# Autodesk Inventor assembly: Test Section Assembly
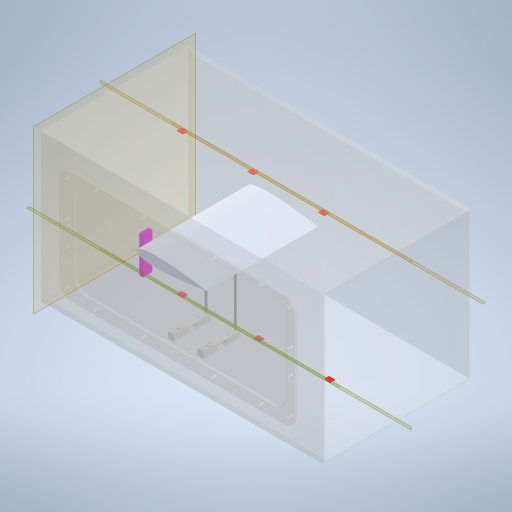
[picture p0: Inventor's stored thumbnail of the model, 512x512]
Saved by Autodesk Inventor 2023 (Build 270158000, 158)
## iProperties
Created: 2022-03-05
Part Number: Test Section Assembly
Document SubType Name: Assembly
Designer: kamer
Author: kamer
## iProperties of the stored document MemberDocs/xAaaaqqaaAaaaaaaaAaaaqncaKc
Created: 2022-03-05
Part Number: Test Section Assembly
Document SubType Name: Assembly
Designer: kamer
Author: kamer
## Documents named in this file (13)
- X:\Storage\Documents\ME 306 Heat Transfer Project Files\CAD\Test Section Assembly.iam
- X:\Storage\Documents\ME 306 Heat Transfer Project Files\CAD\Wind Tunnel Test Section Back.ipt
- X:\Storage\Documents\ME 306 Heat Transfer Project Files\CAD\Wind Tunnel Test Section Bottom.ipt
- X:\Storage\Documents\ME 306 Heat Transfer Project Files\CAD\Wind Tunnel Test Section Front.ipt
- X:\Storage\Documents\ME 306 Heat Transfer Project Files\CAD\Wind Tunnel Test Section Top.ipt
- X:\Storage\Documents\ME 306 Heat Transfer Project Files\CAD\Wind Tunnel Test Section Door Inner.ipt
- X:\Storage\Documents\ME 306 Heat Transfer Project Files\CAD\Wind Tunnel Test Section Door Outer.ipt
- X:\Storage\Documents\ME 306 Heat Transfer Project Files\CAD\Load Cell Spacer.ipt
- X:\Storage\Documents\ME 306 Heat Transfer Project Files\CAD\Mockup Load Cell (based on 1kg Adafruit).ipt
- X:\Storage\Documents\ME 306 Heat Transfer Project Files\CAD\naca0015_airfoil_heatstakes.ipt
- X:\Storage\Documents\ME 306 Heat Transfer Project Files\CAD\4mm threadstock 7in length.ipt
- X:\Storage\Documents\ME 306 Heat Transfer Project Files\CAD\Mockup Barometer.ipt
- X:\Storage\Documents\ME 306 Heat Transfer Project Files\CAD\Mockup Anemometer.ipt
## Components (22 placed, 12 different names)
1. Wind Tunnel Test Section Back:1 — Mate:1, Flush:1, Mate:4, Mate:5, Mate:42
2. Wind Tunnel Test Section Bottom:1 — Mate:1, Flush:1, Mate:2, Flush:2, Mate:10, Mate:15, Mate:16, Mate:21, Mate:22, Mate:23, Mate:35, Mate:36, Mate:37, Mate:38, Mate:39, Mate:40, Mate:41, Flush:14
3. Wind Tunnel Test Section Front:1 — Mate:2, Flush:2, Mate:3, Flush:3, Mate:5, Mate:6, Flush:4, Mate:7, Mate:8, Angle:1, Mate:24, Angle:3, Mate:43
4. Wind Tunnel Test Section Top:1 — Mate:3, Flush:3, Mate:4, Mate:6, Mate:28, Mate:29, Mate:30, Mate:31, Mate:32, Mate:33, Mate:34
5. Wind Tunnel Test Section Door Inner:1 — Flush:4, Mate:7, Mate:8, Mate:9, Flush:5, Flush:6
6. Wind Tunnel Test Section Door Outer:1 — Mate:9, Flush:5, Flush:6
7. Load Cell Spacer:1 — Mate:11, Mate:12, Mate:15
8. Mockup Load Cell (based on 1kg Adafruit):1 — Mate:10, Mate:11, Mate:12, Mate:13, Mate:14, Angle:1, Mate:26, Angle:2
9. Load Cell Spacer:2 — Mate:13, Mate:14
10. Mockup Load Cell (based on 1kg Adafruit):2 — Mate:16, Mate:17, Mate:18, Mate:19, Mate:20, Mate:25, Angle:2
11. Load Cell Spacer:3 — Mate:18, Mate:20, Mate:21
12. Load Cell Spacer:4 — Mate:17, Mate:19
13. naca0015_airfoil_heatstakes:1 — Mate:22, Mate:23, Mate:24, Mate:27
14. 4mm threadstock 7in length:1 — Mate:26, Mate:27, Flush:8
15. 4mm threadstock 7in length:2 — Mate:25, Flush:8
16. Mockup Barometer:1 — Mate:33, Mate:34, Flush:10, Flush:11
17. Mockup Barometer:2 — Mate:36, Mate:37, Flush:12
18. Mockup Barometer:3 — Mate:31, Mate:32, Flush:9, Flush:10, Flush:12
19. Mockup Barometer:4 — Mate:38, Mate:39, Flush:13
20. Mockup Barometer:5 — Mate:28, Mate:29, Mate:30, Flush:9, Flush:13
21. Mockup Barometer:6 — Mate:35, Flush:11, Mate:40
22. Mockup Anemometer:1 — Mate:41, Angle:3, Flush:14, Mate:44
## Relationships (60: Mate 44, Flush 13, Angle 3)
- Mate:1: Wind Tunnel Test Section Back:1 ↔ Wind Tunnel Test Section Bottom:1
- Flush:1: Wind Tunnel Test Section Back:1 ↔ Wind Tunnel Test Section Bottom:1
- Mate:2: Wind Tunnel Test Section Bottom:1 ↔ Wind Tunnel Test Section Front:1
- Flush:2: Wind Tunnel Test Section Bottom:1 ↔ Wind Tunnel Test Section Front:1
- Mate:3: Wind Tunnel Test Section Front:1 ↔ Wind Tunnel Test Section Top:1
- Flush:3: Wind Tunnel Test Section Front:1 ↔ Wind Tunnel Test Section Top:1
- Mate:4: Wind Tunnel Test Section Back:1 ↔ Wind Tunnel Test Section Top:1
- Mate:5 (306.3494 mm): Wind Tunnel Test Section Back:1 ↔ Wind Tunnel Test Section Front:1
- Mate:6: Wind Tunnel Test Section Front:1 ↔ Wind Tunnel Test Section Top:1
- Flush:4: Wind Tunnel Test Section Front:1 ↔ Wind Tunnel Test Section Door Inner:1
- Mate:7: Wind Tunnel Test Section Front:1 ↔ Wind Tunnel Test Section Door Inner:1
- Mate:8: Wind Tunnel Test Section Front:1 ↔ Wind Tunnel Test Section Door Inner:1
- Mate:9: Wind Tunnel Test Section Door Inner:1 ↔ Wind Tunnel Test Section Door Outer:1
- Flush:5 (-26.2763 mm): Wind Tunnel Test Section Door Inner:1 ↔ Wind Tunnel Test Section Door Outer:1
- Flush:6 (-18.2753 mm): Wind Tunnel Test Section Door Inner:1 ↔ Wind Tunnel Test Section Door Outer:1
- Mate:10: Wind Tunnel Test Section Bottom:1 ↔ Mockup Load Cell (based on 1kg Adafruit):1
- Mate:11: Load Cell Spacer:1 ↔ Mockup Load Cell (based on 1kg Adafruit):1
- Mate:12: Load Cell Spacer:1 ↔ Mockup Load Cell (based on 1kg Adafruit):1
- Mate:13: Mockup Load Cell (based on 1kg Adafruit):1 ↔ Load Cell Spacer:2
- Mate:14: Mockup Load Cell (based on 1kg Adafruit):1 ↔ Load Cell Spacer:2
- Mate:15: Wind Tunnel Test Section Bottom:1 ↔ Load Cell Spacer:1
- Angle:1 (270 deg): Wind Tunnel Test Section Front:1 ↔ Mockup Load Cell (based on 1kg Adafruit):1
- Mate:16: Wind Tunnel Test Section Bottom:1 ↔ Mockup Load Cell (based on 1kg Adafruit):2
- Mate:17: Mockup Load Cell (based on 1kg Adafruit):2 ↔ Load Cell Spacer:4
- Mate:18: Mockup Load Cell (based on 1kg Adafruit):2 ↔ Load Cell Spacer:3
- Mate:19: Mockup Load Cell (based on 1kg Adafruit):2 ↔ Load Cell Spacer:4
- Mate:20: Mockup Load Cell (based on 1kg Adafruit):2 ↔ Load Cell Spacer:3
- Mate:21: Wind Tunnel Test Section Bottom:1 ↔ Load Cell Spacer:3
- Mate:22: Wind Tunnel Test Section Bottom:1 ↔ naca0015_airfoil_heatstakes:1
- Mate:23: Wind Tunnel Test Section Bottom:1 ↔ naca0015_airfoil_heatstakes:1
- Mate:24: Wind Tunnel Test Section Front:1 ↔ naca0015_airfoil_heatstakes:1
- Mate:25: Mockup Load Cell (based on 1kg Adafruit):2 ↔ 4mm threadstock 7in length:2
- Mate:26: Mockup Load Cell (based on 1kg Adafruit):1 ↔ 4mm threadstock 7in length:1
- Mate:27: naca0015_airfoil_heatstakes:1 ↔ 4mm threadstock 7in length:1
- Flush:8: 4mm threadstock 7in length:1 ↔ 4mm threadstock 7in length:2
- Mate:28: Wind Tunnel Test Section Top:1 ↔ Mockup Barometer:5
- Mate:29: Wind Tunnel Test Section Top:1 ↔ Mockup Barometer:5
- Mate:30 (-5 mm): Wind Tunnel Test Section Top:1 ↔ Mockup Barometer:5
- Mate:31: Wind Tunnel Test Section Top:1 ↔ Mockup Barometer:3
- Mate:32: Wind Tunnel Test Section Top:1 ↔ Mockup Barometer:3
- Flush:9: Mockup Barometer:3 ↔ Mockup Barometer:5
- Mate:33: Wind Tunnel Test Section Top:1 ↔ Mockup Barometer:1
- Mate:34: Wind Tunnel Test Section Top:1 ↔ Mockup Barometer:1
- Flush:10: Mockup Barometer:1 ↔ Mockup Barometer:3
- Angle:2 (180 deg): Mockup Load Cell (based on 1kg Adafruit):1 ↔ Mockup Load Cell (based on 1kg Adafruit):2
- Mate:35: Wind Tunnel Test Section Bottom:1 ↔ Mockup Barometer:6
- Flush:11: Mockup Barometer:1 ↔ Mockup Barometer:6
- Mate:36: Wind Tunnel Test Section Bottom:1 ↔ Mockup Barometer:2
- Mate:37: Wind Tunnel Test Section Bottom:1 ↔ Mockup Barometer:2
- Flush:12: Mockup Barometer:2 ↔ Mockup Barometer:3
- Mate:38: Wind Tunnel Test Section Bottom:1 ↔ Mockup Barometer:4
- Mate:39: Wind Tunnel Test Section Bottom:1 ↔ Mockup Barometer:4
- Flush:13: Mockup Barometer:4 ↔ Mockup Barometer:5
- Mate:40: Wind Tunnel Test Section Bottom:1 ↔ Mockup Barometer:6
- Mate:41: Wind Tunnel Test Section Bottom:1 ↔ Mockup Anemometer:1
- Angle:3 (90 deg): Wind Tunnel Test Section Front:1 ↔ Mockup Anemometer:1
- Flush:14 (-10 mm): Wind Tunnel Test Section Bottom:1 ↔ Mockup Anemometer:1
- Mate:42: Wind Tunnel Test Section Back:1
- Mate:43: Wind Tunnel Test Section Front:1
- Mate:44 (63.5 mm): Mockup Anemometer:1
